# Autodesk Inventor assembly: Bridge
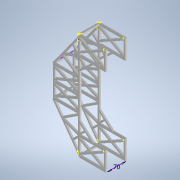
[picture p0: Inventor's stored thumbnail of the model, 180x180]
Saved by Autodesk Inventor 2020.1 (Build 241239000, 239)
## iProperties
Created: 2020-02-04
Part Number: Bridge
Document SubType Name: Assembly
Designer: super
Author: super
## Documents named in this file (14)
- C:\Users\super\Desktop\Giovanni\Science\3D Models\Autodesk-Inventor\Projects\FAS\Bridge.iam
- C:\Users\super\Desktop\Giovanni\Science\3D Models\Autodesk-Inventor\Projects\FAS\BottomBottom.ipt
- C:\Users\super\Desktop\Giovanni\Science\3D Models\Autodesk-Inventor\Projects\FAS\BottomDiagonalSupport.ipt
- C:\Users\super\Desktop\Giovanni\Science\3D Models\Autodesk-Inventor\Projects\FAS\BottomSquareSupport.ipt
- C:\Users\super\Desktop\Giovanni\Science\3D Models\Autodesk-Inventor\Projects\FAS\InnerDiagonalSupport.ipt
- C:\Users\super\Desktop\Giovanni\Science\3D Models\Autodesk-Inventor\Projects\FAS\Main.ipt
- C:\Users\super\Desktop\Giovanni\Science\3D Models\Autodesk-Inventor\Projects\FAS\UpperExteriorDiagonal.ipt
- C:\Users\super\Desktop\Giovanni\Science\3D Models\Autodesk-Inventor\Projects\FAS\UpperMiniSupport.ipt
- C:\Users\super\Desktop\Giovanni\Science\3D Models\Autodesk-Inventor\Projects\FAS\TopTop.ipt
- C:\Users\super\Desktop\Giovanni\Science\3D Models\Autodesk-Inventor\Projects\FAS\UpperInnerWD1.ipt
- C:\Users\super\Desktop\Giovanni\Science\3D Models\Autodesk-Inventor\Projects\FAS\UpperInnerWD2.ipt
- C:\Users\super\Desktop\Giovanni\Science\3D Models\Autodesk-Inventor\Projects\FAS\UpperSquareSupport.ipt
- C:\Users\super\Desktop\Giovanni\Science\3D Models\Autodesk-Inventor\Projects\FAS\UpperInnerDiagonal.ipt
- C:\Users\super\Desktop\Giovanni\Science\3D Models\Autodesk-Inventor\Projects\FAS\Connectors.ipt
## Components (66 placed, 13 different names)
1. BottomBottom:1 — Mate:1, Flush:1, Flush:2, Flush:3, Mate:2, Flush:4, Mate:3, Flush:15, Mate:12
2. BottomDiagonalSupport:1 — Mate:3, Mate:12
3. BottomSquareSupport:1 — Mate:1, Flush:1, Flush:2, Flush:16, Flush:17
4. BottomSquareSupport:2 — Flush:3, Mate:2, Flush:4, Flush:19, Mate:16
5. BottomDiagonalSupport:2
6. BottomBottom:2 — Flush:15
7. BottomDiagonalSupport:3
8. BottomSquareSupport:3 — Mate:11, Mate:14
9. BottomSquareSupport:4 — Flush:18, Flush:19
10. BottomDiagonalSupport:4
11. Main:1 — Flush:16, Flush:17, Flush:18, Mate:11, Mate:13, Flush:25, Mate:15, Flush:26, Mate:19
12. InnerDiagonalSupport:1 — Mate:13, Mate:14, Flush:25
13. InnerDiagonalSupport:2 — Mate:15, Mate:16, Flush:26
14. UpperExteriorDiagonal:1
15. UpperExteriorDiagonal:2
16. UpperMiniSupport:1 — Mate:19
17. UpperMiniSupport:2
18. UpperMiniSupport:3
19. UpperMiniSupport:4
20. TopTop:1
21. UpperInnerWD1:1
22. UpperInnerWD1:2
23. UpperInnerWD2:1
24. UpperInnerWD2:2
25. UpperSquareSupport:1
26. UpperSquareSupport:2
27. UpperSquareSupport:3
28. UpperInnerDiagonal:1
29. UpperInnerDiagonal:2
30. UpperInnerDiagonal:3
31. UpperInnerDiagonal:4
32. BottomBottom:3
33. BottomDiagonalSupport:5
34. BottomSquareSupport:5
35. BottomSquareSupport:6
36. BottomDiagonalSupport:6
37. BottomBottom:4
38. BottomDiagonalSupport:7
39. BottomSquareSupport:7
40. BottomSquareSupport:8
41. BottomDiagonalSupport:8
42. Main:2
43. InnerDiagonalSupport:3
44. InnerDiagonalSupport:4
45. UpperExteriorDiagonal:3
46. UpperExteriorDiagonal:4
47. UpperMiniSupport:5
48. UpperMiniSupport:6
49. UpperMiniSupport:7
50. UpperMiniSupport:8
51. TopTop:2
52. UpperInnerWD1:3
53. UpperInnerWD1:4
54. UpperInnerWD2:3
55. UpperInnerWD2:4
56. UpperSquareSupport:4
57. UpperSquareSupport:5
58. UpperSquareSupport:6
59. UpperInnerDiagonal:5
60. UpperInnerDiagonal:6
61. UpperInnerDiagonal:7
62. UpperInnerDiagonal:8
63. Connectors:1
64. Connectors:2
65. Connectors:3
66. Connectors:4
## Relationships (68: Flush 36, Mate 30, WeldJoint 2)
- Mate:1: BottomBottom:1 ↔ BottomSquareSupport:1
- Flush:1: BottomBottom:1 ↔ BottomSquareSupport:1
- Flush:2: BottomBottom:1 ↔ BottomSquareSupport:1
- Flush:3: BottomBottom:1 ↔ BottomSquareSupport:2
- Mate:2: BottomBottom:1 ↔ BottomSquareSupport:2
- Flush:4: BottomBottom:1 ↔ BottomSquareSupport:2
- Mate:3: BottomBottom:1 ↔ BottomDiagonalSupport:1
- [Mate]: BottomBottom:2 ↔ BottomSquareSupport:3
- [Flush]: BottomBottom:2 ↔ BottomSquareSupport:3
- [Flush]: BottomBottom:2 ↔ BottomSquareSupport:3
- [Flush]: BottomBottom:2 ↔ BottomSquareSupport:4
- [Mate]: BottomBottom:2 ↔ BottomSquareSupport:4
- [Flush]: BottomBottom:2 ↔ BottomSquareSupport:4
- [Mate]: BottomBottom:2 ↔ BottomDiagonalSupport:3
- [Flush]: BottomBottom:2 ↔ BottomDiagonalSupport:4
- [Mate]: BottomBottom:2 ↔ BottomDiagonalSupport:4
- [WeldJoint]: BottomSquareSupport:4 ↔ BottomDiagonalSupport:4
- [Mate]: BottomBottom:2 ↔ BottomDiagonalSupport:4
- [Flush]: BottomBottom:2 ↔ BottomDiagonalSupport:4
- [Flush]: BottomDiagonalSupport:3 ↔ BottomDiagonalSupport:4
- Flush:15: BottomBottom:1 ↔ BottomBottom:2
- Flush:16: BottomSquareSupport:1 ↔ Main:1
- Flush:17: BottomSquareSupport:1 ↔ Main:1
- Flush:18: BottomSquareSupport:4 ↔ Main:1
- Mate:11: BottomSquareSupport:3 ↔ Main:1
- Flush:19: BottomSquareSupport:2 ↔ BottomSquareSupport:4
- Mate:12: BottomBottom:1 ↔ BottomDiagonalSupport:1
- Mate:13: Main:1 ↔ InnerDiagonalSupport:1
- Mate:14: BottomSquareSupport:3 ↔ InnerDiagonalSupport:1
- Flush:25: Main:1 ↔ InnerDiagonalSupport:1
- Mate:15: Main:1 ↔ InnerDiagonalSupport:2
- Mate:16: BottomSquareSupport:2 ↔ InnerDiagonalSupport:2
- Flush:26: Main:1 ↔ InnerDiagonalSupport:2
- Mate:19: Main:1 ↔ UpperMiniSupport:1
- [Mate]: BottomBottom:3 ↔ BottomSquareSupport:5
- [Flush]: BottomBottom:3 ↔ BottomSquareSupport:5
- [Flush]: BottomBottom:3 ↔ BottomSquareSupport:5
- [Flush]: BottomBottom:3 ↔ BottomSquareSupport:6
- [Mate]: BottomBottom:3 ↔ BottomSquareSupport:6
- [Flush]: BottomBottom:3 ↔ BottomSquareSupport:6
- [Mate]: BottomBottom:3 ↔ BottomDiagonalSupport:5
- [Mate]: BottomBottom:4 ↔ BottomSquareSupport:7
- [Flush]: BottomBottom:4 ↔ BottomSquareSupport:7
- [Flush]: BottomBottom:4 ↔ BottomSquareSupport:7
- [Flush]: BottomBottom:4 ↔ BottomSquareSupport:8
- [Mate]: BottomBottom:4 ↔ BottomSquareSupport:8
- [Flush]: BottomBottom:4 ↔ BottomSquareSupport:8
- [Mate]: BottomBottom:4 ↔ BottomDiagonalSupport:7
- [Flush]: BottomBottom:4 ↔ BottomDiagonalSupport:8
- [Mate]: BottomBottom:4 ↔ BottomDiagonalSupport:8
- [WeldJoint]: BottomSquareSupport:8 ↔ BottomDiagonalSupport:8
- [Mate]: BottomBottom:4 ↔ BottomDiagonalSupport:8
- [Flush]: BottomBottom:4 ↔ BottomDiagonalSupport:8
- [Flush]: BottomDiagonalSupport:7 ↔ BottomDiagonalSupport:8
- [Flush]: BottomBottom:3 ↔ BottomBottom:4
- [Flush]: BottomSquareSupport:5 ↔ Main:2
- [Flush]: BottomSquareSupport:5 ↔ Main:2
- [Flush]: BottomSquareSupport:8 ↔ Main:2
- [Mate]: BottomSquareSupport:7 ↔ Main:2
- [Flush]: BottomSquareSupport:6 ↔ BottomSquareSupport:8
- [Mate]: BottomBottom:3 ↔ BottomDiagonalSupport:5
- [Mate]: Main:2 ↔ InnerDiagonalSupport:3
- [Mate]: BottomSquareSupport:7 ↔ InnerDiagonalSupport:3
- [Flush]: Main:2 ↔ InnerDiagonalSupport:3
- [Mate]: Main:2 ↔ InnerDiagonalSupport:4
- [Mate]: BottomSquareSupport:6 ↔ InnerDiagonalSupport:4
- [Flush]: Main:2 ↔ InnerDiagonalSupport:4
- [Mate]: Main:2 ↔ UpperMiniSupport:5
## Named parameters: d13_d10 = 0 mm, d14_d11 = 0 mm, d15_d12 = 0 mm, d16_d1 = 0 mm, d17_d2 = 0 mm, d18_d3 = 0 mm, d19_d4 = 0 mm, d20_d5 = 0 mm, d21_d6 = 0 mm, d22_d7 = 0 mm, d23_d8 = 0 mm, d24_d9 = 0 mm, d25_d0 = 0 mm, d90_d39 = 0 mm, d91_d40 = 0 mm, d92_d41 = 0 mm, d93_d42 = 0 mm, d94_d43 = 0 mm, d95_d44 = 0 mm, d96_d49 = 0 mm, d97_d6 = 0 mm, d98_d13_d10 = 0 mm, d99_d14_d11 = 0 mm, d100_d15_d12 = 0 mm, d101_d16_d1 = 0 mm, d102_d17_d2 = 0 mm, d103_d18_d3 = 0 mm, d104_d19_d4 = 0 mm, d105_d20_d5 = 0 mm, d106_d21_d6 = 0 mm, d107_d22_d7 = 0 mm, d108_d23_d8 = 0 mm, d109_d24_d9 = 0 mm, d110_d25_d0 = 0 mm, d111_d26 = 0 mm, d112_d27 = 0 mm, d113_d28 = 0 mm, d114_d29 = 0 mm, d115_d30 = 0 mm, d116_d31 = 0 mm, d117_d32 = 0 mm, d118_d0 = 0 mm, d119_d1 = 0 mm, d120_d2 = 0 mm, d121_d3 = 0 mm, d122_d4 = 0 mm, d123_d5 = 0 mm
